# Autodesk Inventor assembly: Housing 3
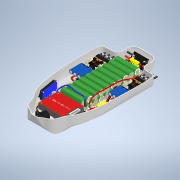
[picture p0: Inventor's stored thumbnail of the model, 180x180]
Saved by Autodesk Inventor 2020.1 (Build 241239000, 239)
## iProperties
Created: 2019-07-26
Part Number: Housing 3
Document SubType Name: Assembly
Designer: Petar
Author: Petar
## Documents named in this file (12)
- D:\OMG\E-Board\CAD\Inventor\Housing\Housing 3.iam
- D:\OMG\E-Board\CAD\Inventor\Housing\Battery Housing Box v2.ipt
- D:\OMG\E-Board\CAD\Inventor\Electrical Components\Battery Indicator.ipt
- D:\OMG\E-Board\CAD\Inventor\Electrical Components\Power Button.ipt
- D:\OMG\E-Board\CAD\Inventor\Electrical Components\VESC - detail.ipt
- D:\OMG\E-Board\CAD\Inventor\Electrical Components\XLR Female Plug.ipt
- D:\OMG\E-Board\CAD\Inventor\Electrical Components\Battery Pack\Samsung 25R\Battery Pack - Samsung 25R - 2xRows.iam
- D:\OMG\E-Board\CAD\Inventor\Electrical Components\Power Switch - detail.ipt
- D:\OMG\E-Board\CAD\Inventor\Remote\Receiver.iam
- D:\OMG\E-Board\CAD\Inventor\Electrical Components\XT60\XT60 Connectors.iam
- D:\OMG\E-Board\CAD\Inventor\Electrical Components\BMS (separate port).ipt
- D:\OMG\E-Board\CAD\Inventor\Housing\Cable and Harness\Housing 3.Harness1.iam
## Components (15 placed, 11 different names)
1. Receiver:1 [sub-assembly]
2. Battery Housing Box v2:1 — Flush:3
3. Battery Indicator:1
4. BMS (separate port):1
5. Power Button:1
6. XLR Female Plug:1 — Flush:3
7. VESC - detail:2 — Flush:1, Flush:2
8. Battery Pack - Samsung 25R - 2xRows:1 [sub-assembly]
9. Power Switch - detail:1
10. VESC - detail:3 — Flush:1, Flush:2
11. XT60 Connectors:2 [sub-assembly]
12. XT60 Connectors:4 [sub-assembly]
13. XT60 Connectors:5 [sub-assembly]
14. XT60 Connectors:6 [sub-assembly]
15. Harness1 [sub-assembly]
## Relationships (3: Flush 3)
- Flush:1: VESC - detail:2 ↔ VESC - detail:3
- Flush:2: VESC - detail:2 ↔ VESC - detail:3
- Flush:3 (-2 mm): Battery Housing Box v2:1 ↔ XLR Female Plug:1
